# Autodesk Inventor assembly: 4in Performance Bearings
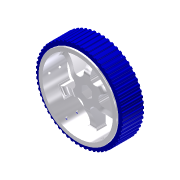
[picture p0: Inventor's stored thumbnail of the model, 180x180]
Saved by Autodesk Inventor 2011 (Build 150239000, 239)
## iProperties
Created: 2012-06-01
Part Number: 4in Performance Bearings
Document SubType Name: Assembly
Designer: Nemo
Author: Nemo
## Documents named in this file (3)
- H:\Nemo\Documents\Robotics\COTS Parts\Wheels\4in Performance Hex Bore.iam
- H:\Nemo\Documents\Robotics\COTS Parts\Wheels\Performance Wheel Parts\Nitrile Tread.ipt
- H:\Nemo\Documents\Robotics\COTS Parts\Wheels\Performance Wheel Parts\4in Performance Hex.ipt
## Components (2 placed, 2 different names)
1. 4in Performance Hex:1 — Insert:1
2. Nitrile Tread:1 — Insert:1
## Relationships (1: Insert 1)
- Insert:1: 4in Performance Hex:1 ↔ Nitrile Tread:1
